# Autodesk Inventor assembly: robot arm box
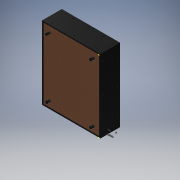
[picture p0: Inventor's stored thumbnail of the model, 180x180]
Saved by Autodesk Inventor 2018 (Build 220112000, 112)
## iProperties
Created: 2017-10-09
Part Number: robot arm box
Document SubType Name: Assembly
Designer: HP
Author: HP
## Documents named in this file (9)
- C:\!_Dani\!_cloud\ownCloud\rover\Robot arm box\robot arm box.iam
- C:\!_Dani\!_cloud\ownCloud\rover\Robot arm box\basic plate.ipt
- C:\!_Dani\!_cloud\ownCloud\rover\Robot arm box\sides.ipt
- C:\!_Dani\!_cloud\ownCloud\rover\Robot arm box\fronts.ipt
- C:\Users\HP\Documents\Inventor\Content Center Files\R2018\en-US\ISO 7046-1 Z(1)\ISO 7046-1 - M3 x 12 - 4.8 - Z - ISO.ipt
- C:\Users\HP\Documents\Inventor\Content Center Files\R2018\en-US\JIS B 1122 - C-Z(2)\JIS B 1122 - ST4,8 x 19 - C - Z(1).ipt
- C:\Users\HP\Documents\Inventor\Content Center Files\R2018\en-US\ISO 4032(2)\ISO 4032 - M3 - ISO.ipt
- C:\!_Dani\!_cloud\ownCloud\rover\Robot arm box\top.ipt
- C:\!_Dani\!_cloud\ownCloud\rover\Robot arm box\robot arm box parameters.xlsx
## Components (9 placed, 7 different names)
1. basic plate:1 — Flush:2, Mate:1, Mate:2, Flush:3, Flush:4, Flush:5, Flush:8, Mate:3, Flush:10, Flush:13
2. sides:1 — Flush:3, Flush:4, Flush:6
3. sides:2 — Flush:5, Flush:6, Mate:3, Flush:9, Flush:12, Flush:14
4. fronts:1 — Flush:8, Flush:9, Flush:11, Flush:13
5. fronts:2 — Flush:10, Flush:11, Flush:12
6. ISO 7046-1 Z M3 x 12 - 4.8 - Z:1
7. JIS B 1122 - C-Z ST4,8 x 19 - C - Z:1
8. ISO 4032 M3:1
9. top:1 — Flush:14
## Relationships (15: Flush 12, Mate 3)
- Flush:2: basic plate:1
- Mate:1: basic plate:1
- Mate:2: basic plate:1
- Flush:3: basic plate:1 ↔ sides:1
- Flush:4 (0.5 mm): basic plate:1 ↔ sides:1
- Flush:5: basic plate:1 ↔ sides:2
- Flush:6: sides:1 ↔ sides:2
- Flush:8: basic plate:1 ↔ fronts:1
- Mate:3 (0.5 mm): basic plate:1 ↔ sides:2
- Flush:9: sides:2 ↔ fronts:1
- Flush:10: basic plate:1 ↔ fronts:2
- Flush:11: fronts:1 ↔ fronts:2
- Flush:12: sides:2 ↔ fronts:2
- Flush:13: basic plate:1 ↔ fronts:1
- Flush:14: sides:2 ↔ top:1
## Named parameters: plate_thickness = 5 mm, ABS_tolerance = 0.1 mm, laser_cutter_thickness = 0.1 mm, basic_plate_offset = 0.5 mm
